# Autodesk Inventor assembly: layer2
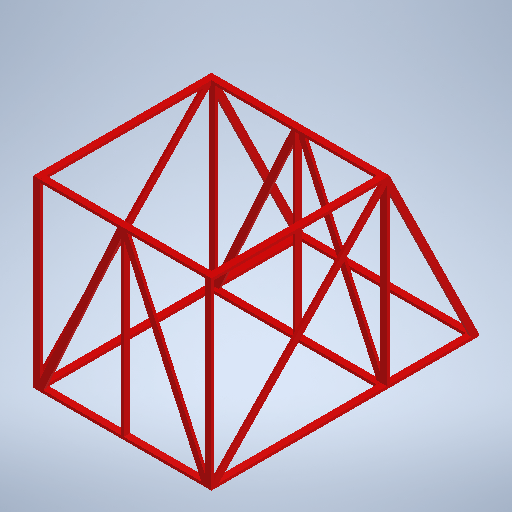
[picture p0: Inventor's stored thumbnail of the model, 512x512]
Saved by Autodesk Inventor 2025.1 (Build 291241020, 241B)
## iProperties
Created: 2024-09-19
Part Number: layer2
Document SubType Name: Assembly
Designer: User
Author: User
## Documents named in this file (7)
- C:\Users\User\Documents\Tburn24\layer2\layer2.iam
- C:\Users\User\Documents\Tburn24\layer2\12'x2x4.ipt
- C:\Users\User\Documents\Tburn24\layer2\7'5x2x4.ipt
- C:\Users\User\Documents\Tburn24\layer2\8'x2x4.ipt
- C:\Users\User\Documents\Tburn24\layer2\s48x2x4b.ipt
- C:\Users\User\Documents\Tburn24\layer2\s88x2x4.ipt
- C:\Users\User\Documents\Tburn24\layer2\s48x2x4a.ipt
## Components (23 placed, 6 different names)
1. 12'x2x4:1 — Flush:3, Flush:4, Flush:5, Mate:2, Mate:3, Mate:5, Flush:15, Flush:16, Flush:17, Flush:38
2. 12'x2x4:2 — Flush:3, Flush:4, Flush:5, Mate:1, Flush:6, Flush:7, Flush:8, Flush:9, Flush:10, Mate:4, Mate:6, Flush:12, Flush:13, Flush:14, Mate:24
3. 7'5x2x4:1 — Mate:1, Flush:6, Flush:7, Flush:11, Mate:12, Flush:29
4. 7'5x2x4:2 — Flush:10, Flush:11, Flush:18, Flush:19, Mate:11, Flush:28
5. 7'5x2x4:3 — Flush:8, Flush:9, Mate:2
6. 8'x2x4:1 — Mate:4, Flush:13, Flush:14, Mate:8, Flush:21, Flush:22, Flush:36
7. 8'x2x4:2 — Mate:3, Flush:15, Flush:16, Mate:7, Flush:20, Flush:23, Flush:30
8. 8'x2x4:3 — Mate:5, Flush:17, Flush:18, Flush:31, Mate:22
9. 8'x2x4:4 — Mate:6, Flush:12, Flush:19, Mate:23, Flush:39
10. 8'x2x4:5 — Mate:8, Flush:21, Flush:22, Mate:9, Flush:26, Mate:10, Flush:27
11. 8'x2x4:6 — Mate:7, Flush:20, Flush:23, Flush:24, Flush:25, Mate:21, Flush:37
12. 7'5x2x4:4 — Flush:24, Mate:10, Flush:27, Mate:14, Mate:16
13. 7'5x2x4:5 — Flush:25, Mate:9, Flush:26, Mate:18, Mate:20
14. 8'x2x4:7 — Mate:12, Flush:29, Flush:30, Mate:13, Flush:32, Mate:15, Flush:33
15. 8'x2x4:8 — Mate:11, Flush:28, Flush:31, Mate:17, Flush:34, Mate:19, Flush:35
16. s48x2x4b:1 — Mate:13, Mate:14, Flush:32
17. s48x2x4b:2 — Mate:15, Mate:16, Flush:33
18. s48x2x4b:3 — Mate:17, Mate:18, Flush:34
19. s48x2x4b:4 — Mate:19, Mate:20, Flush:35
20. s88x2x4:1 — Flush:36
21. s88x2x4:2 — Mate:21, Mate:22, Flush:37
22. s48x2x4a:1 — Flush:38
23. s48x2x4a:2 — Mate:23, Mate:24, Flush:39
## Relationships (61: Flush 37, Mate 24)
- Flush:3 (2349.5 mm): 12'x2x4:1 ↔ 12'x2x4:2
- Flush:4: 12'x2x4:1 ↔ 12'x2x4:2
- Flush:5: 12'x2x4:1 ↔ 12'x2x4:2
- Mate:1: 12'x2x4:2 ↔ 7'5x2x4:1
- Flush:6: 12'x2x4:2 ↔ 7'5x2x4:1
- Flush:7: 12'x2x4:2 ↔ 7'5x2x4:1
- Flush:8: 12'x2x4:2 ↔ 7'5x2x4:3
- Flush:9: 12'x2x4:2 ↔ 7'5x2x4:3
- Mate:2: 12'x2x4:1 ↔ 7'5x2x4:3
- Flush:10: 12'x2x4:2 ↔ 7'5x2x4:2
- Flush:11 (2349.5 mm): 7'5x2x4:1 ↔ 7'5x2x4:2
- Mate:3: 12'x2x4:1 ↔ 8'x2x4:2
- Mate:4: 12'x2x4:2 ↔ 8'x2x4:1
- Mate:5: 12'x2x4:1 ↔ 8'x2x4:3
- Mate:6: 12'x2x4:2 ↔ 8'x2x4:4
- Flush:12: 12'x2x4:2 ↔ 8'x2x4:4
- Flush:13: 12'x2x4:2 ↔ 8'x2x4:1
- Flush:14: 12'x2x4:2 ↔ 8'x2x4:1
- Flush:15: 12'x2x4:1 ↔ 8'x2x4:2
- Flush:16: 12'x2x4:1 ↔ 8'x2x4:2
- Flush:17: 12'x2x4:1 ↔ 8'x2x4:3
- Flush:18: 7'5x2x4:2 ↔ 8'x2x4:3
- Flush:19: 7'5x2x4:2 ↔ 8'x2x4:4
- Mate:7: 8'x2x4:2 ↔ 8'x2x4:6
- Mate:8: 8'x2x4:1 ↔ 8'x2x4:5
- Flush:20: 8'x2x4:2 ↔ 8'x2x4:6
- Flush:21: 8'x2x4:1 ↔ 8'x2x4:5
- Flush:22: 8'x2x4:1 ↔ 8'x2x4:5
- Flush:23: 8'x2x4:2 ↔ 8'x2x4:6
- Flush:24: 8'x2x4:6 ↔ 7'5x2x4:4
- Flush:25: 8'x2x4:6 ↔ 7'5x2x4:5
- Mate:9: 8'x2x4:5 ↔ 7'5x2x4:5
- Flush:26: 8'x2x4:5 ↔ 7'5x2x4:5
- Mate:10: 8'x2x4:5 ↔ 7'5x2x4:4
- Flush:27: 8'x2x4:5 ↔ 7'5x2x4:4
- Mate:11: 7'5x2x4:2 ↔ 8'x2x4:8
- Flush:28: 7'5x2x4:2 ↔ 8'x2x4:8
- Mate:12: 7'5x2x4:1 ↔ 8'x2x4:7
- Flush:29: 7'5x2x4:1 ↔ 8'x2x4:7
- Flush:30 (1200.15 mm): 8'x2x4:2 ↔ 8'x2x4:7
- Flush:31 (1200.15 mm): 8'x2x4:3 ↔ 8'x2x4:8
- Mate:13: 8'x2x4:7 ↔ s48x2x4b:1
- Mate:14: 7'5x2x4:4 ↔ s48x2x4b:1
- Flush:32: 8'x2x4:7 ↔ s48x2x4b:1
- Mate:15: 8'x2x4:7 ↔ s48x2x4b:2
- Mate:16: 7'5x2x4:4 ↔ s48x2x4b:2
- Flush:33: 8'x2x4:7 ↔ s48x2x4b:2
- Mate:17: 8'x2x4:8 ↔ s48x2x4b:3
- Mate:18: 7'5x2x4:5 ↔ s48x2x4b:3
- Flush:34: 8'x2x4:8 ↔ s48x2x4b:3
- Mate:19: 8'x2x4:8 ↔ s48x2x4b:4
- Mate:20: 7'5x2x4:5 ↔ s48x2x4b:4
- Flush:35: 8'x2x4:8 ↔ s48x2x4b:4
- Flush:36: 8'x2x4:1 ↔ s88x2x4:1
- Mate:21: 8'x2x4:6 ↔ s88x2x4:2
- Mate:22: 8'x2x4:3 ↔ s88x2x4:2
- Flush:37: 8'x2x4:6 ↔ s88x2x4:2
- Flush:38: 12'x2x4:1 ↔ s48x2x4a:1
- Mate:23: 8'x2x4:4 ↔ s48x2x4a:2
- Mate:24: 12'x2x4:2 ↔ s48x2x4a:2
- Flush:39: 8'x2x4:4 ↔ s48x2x4a:2
